# Autodesk Inventor assembly: assem_linact_only
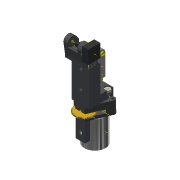
[picture p0: Inventor's stored thumbnail of the model, 180x180]
Saved by Autodesk Inventor 2014 (Build 180170000, 170)
## iProperties
Created: 2015-05-04
Part Number: assem_linact_only
Document SubType Name: Assembly
Designer: Martin
Author: Martin
## Documents named in this file (16)
- C:\Users\Martin\Dropbox\biohand-mec\biohand_v1\fingers\index\assem_linact_only.iam
- C:\Users\Martin\Dropbox\biohand-mec\biohand_v1\fingers\index\linact_knuckle_v2.ipt
- C:\Users\Martin\Dropbox\biohand-mec\biohand_v1\fingers\index\assem_linact_rod_v3.iam
- C:\Users\Martin\Dropbox\biohand-mec\biohand_v1\misc\servo_square_pot.ipt
- C:\Users\Martin\Dropbox\biohand-mec\biohand_v1\misc\bearing_10_4_3.ipt
- C:\Users\Martin\Dropbox\biohand-mec\biohand_v1\misc\m3_25_screw.ipt
- C:\Users\Martin\Dropbox\biohand-mec\biohand_v1\misc\m3_nut.ipt
- C:\Users\Martin\Dropbox\biohand-mec\biohand_v1\misc\servo_gear_2.ipt
- C:\Users\Martin\Dropbox\biohand-mec\biohand_v1\fingers\index\linact_top.ipt
- C:\Users\Martin\Dropbox\biohand-mec\biohand_v1\fingers\index\linact_base.ipt
- C:\Users\Martin\Dropbox\biohand-mec\biohand_v1\misc\m2_8_screw.ipt
- C:\Users\Martin\Dropbox\biohand-mec\biohand_v1\misc\motor_servo.ipt
- C:\Users\Martin\Dropbox\biohand-mec\biohand_v1\misc\m2_4_screw.ipt
- C:\Users\Martin\Dropbox\biohand-mec\biohand_v1\misc\servo_gear_1.ipt
- C:\Users\Martin\Dropbox\biohand-mec\biohand_v1\misc\m2_nut.ipt
- C:\Users\Martin\Dropbox\biohand-mec\biohand_v1\misc\servo_large_dowel.ipt
## Components (18 placed, 15 different names)
1. linact_knuckle_v2:1 — Mate:1, Mate:2, Insert:3, Insert:6, Mate:6, Mate:7, Mate:8, Insert:12
2. assem_linact_rod_v3:1 [sub-assembly] — Mate:1, Mate:2
3. servo_square_pot:1 — Insert:3, Angle:1
4. bearing_10_4_3:1 — Insert:6, Insert:8
5. m3_25_screw:1 — Insert:7
6. m3_nut:1 — Mate:5, Insert:8
7. servo_gear_2:1 — Mate:5, Insert:7
8. linact_top:1 — Mate:6, Mate:7, Mate:8, Mate:9, Mate:10, Mate:11, Insert:13, Insert:21, Insert:22
9. linact_base:1 — Mate:9, Mate:10, Mate:11, Insert:11, Insert:20, Mate:12, Insert:25
10. motor_servo:1 — Insert:11, Angle:3
11. m2_4_screw:1 — Insert:12
12. servo_gear_1:1 — Insert:13
13. m3_nut:2 — Insert:20, Mate:12
14. m2_8_screw:1 — Insert:22, Insert:24
15. m2_8_screw:2 — Insert:21, Insert:23
16. m2_nut:1 — Insert:23
17. m2_nut:2 — Insert:24
18. servo_large_dowel:1 — Insert:25
## Relationships (25: Insert 13, Mate 10, Angle 2)
- Mate:1: linact_knuckle_v2:1 ↔ assem_linact_rod_v3:1
- Mate:2 (0.2 mm): linact_knuckle_v2:1 ↔ assem_linact_rod_v3:1
- Insert:3: linact_knuckle_v2:1 ↔ servo_square_pot:1
- Angle:1 (180 deg): servo_square_pot:1
- Insert:6: linact_knuckle_v2:1 ↔ bearing_10_4_3:1
- Mate:5: m3_nut:1 ↔ servo_gear_2:1
- Insert:7: m3_25_screw:1 ↔ servo_gear_2:1
- Insert:8: bearing_10_4_3:1 ↔ m3_nut:1
- Mate:6: linact_knuckle_v2:1 ↔ linact_top:1
- Mate:7: linact_knuckle_v2:1 ↔ linact_top:1
- Mate:8: linact_knuckle_v2:1 ↔ linact_top:1
- Mate:9: linact_top:1 ↔ linact_base:1
- Mate:10: linact_top:1 ↔ linact_base:1
- Mate:11: linact_top:1 ↔ linact_base:1
- Insert:11: linact_base:1 ↔ motor_servo:1
- Angle:3 (0 deg): motor_servo:1
- Insert:12: linact_knuckle_v2:1 ↔ m2_4_screw:1
- Insert:13 (0.3 mm): linact_top:1 ↔ servo_gear_1:1
- Insert:20: linact_base:1 ↔ m3_nut:2
- Mate:12: linact_base:1 ↔ m3_nut:2
- Insert:21: linact_top:1 ↔ m2_8_screw:2
- Insert:22: linact_top:1 ↔ m2_8_screw:1
- Insert:23: m2_8_screw:2 ↔ m2_nut:1
- Insert:24: m2_8_screw:1 ↔ m2_nut:2
- Insert:25: linact_base:1 ↔ servo_large_dowel:1
